# Autodesk Inventor assembly: Zlozenie
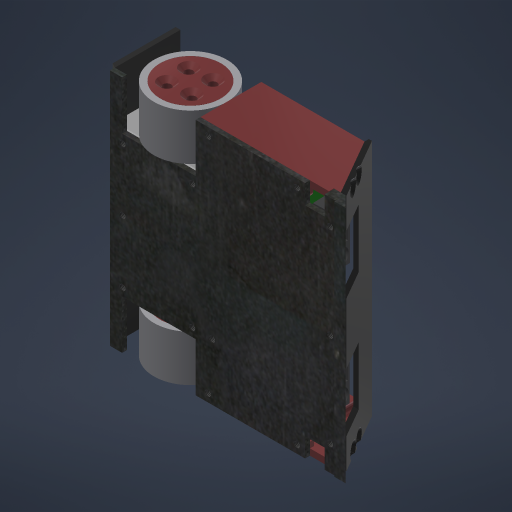
[picture p0: Inventor's stored thumbnail of the model, 512x512]
Saved by Autodesk Inventor 2023 (Build 270158000, 158)
## iProperties
Created: 2021-12-21
Part Number: Zlozenie
Material: Ogólny
Document SubType Name: Assembly
Designer: Michał
Mass: 427.985 g
Surface Area: 1162 cm^2
Volume: 132.956 cm^3
Density: 3.21899 g/cm^3
Author: Michał
## Documents named in this file (13)
- D:\Projekty\RoboIlo\Ser\3D\3D\Zlozenie.iam
- D:\Projekty\RoboIlo\Ser\3D\3D\Blacha.ipt
- D:\Projekty\RoboIlo\Ser\3D\3D\Plug2.ipt
- D:\Projekty\RoboIlo\Ser\3D\3D\Lewybok.ipt
- D:\Projekty\RoboIlo\Ser\3D\3D\Prawybok.ipt
- D:\Projekty\RoboIlo\Ser\3D\3D\Przod.ipt
- D:\Projekty\RoboIlo\Ser\3D\3D\Silnik.ipt
- D:\Projekty\RoboIlo\Ser\3D\3D\sds02a-with-sensor.ipt
- D:\Projekty\RoboIlo\Ser\3D\3D\Tyl.ipt
- D:\Projekty\RoboIlo\Ser\3D\3D\PrzekladniaLewa.iam
- D:\Projekty\RoboIlo\Ser\3D\3D\Kolo.iam
- D:\Projekty\RoboIlo\Ser\3D\3D\PrzekladniaPrawa.iam
- D:\Projekty\RoboIlo\Ser\3D\3D\Dach.ipt
## Components (15 placed, 12 different names)
1. Blacha:1 — Wstaw:1, Wstaw:2, Wstaw:19, Wstaw:20, Wstaw:21, Wstaw:22, Wstaw:36, Wstaw:37, Wstaw:43
2. Plug2:1 — Wstaw:1, Wstaw:2
3. Lewybok:1 — Wstaw:15, Zestawiający:9, Wstaw:19, Wstaw:20, Flush:1
4. Prawybok:1 — Wstaw:16, Zestawiający:10, Wstaw:17, Wstaw:18, Wstaw:21, Wstaw:22
5. Przod:1 — Wstaw:17, Wstaw:18
6. Silnik:1 — Wstaw:38, Wstaw:39
7. Silnik:2 — Wstaw:42
8. sds02a-with-sensor:1 — Wstaw:15, Zestawiający:9
9. sds02a-with-sensor:2 — Wstaw:16, Zestawiający:10
10. Tyl:1
11. PrzekladniaLewa:1 [sub-assembly] — Wstaw:36, Wstaw:37, Wstaw:38, Wstaw:39, Zestawiający:14, Zestawiający:15
12. Kolo:1 [sub-assembly] — Zestawiający:14, Zestawiający:15
13. PrzekladniaPrawa:1 [sub-assembly] — Wstaw:42, Wstaw:43, Zestawiający:16, Zestawiający:17
14. Kolo:2 [sub-assembly] — Zestawiający:16, Zestawiający:17
15. Dach:1 — Flush:1
## Relationships (23: Insert 16, Mate 6, Flush 1)
- Wstaw:1 [Insert]: Blacha:1 ↔ Plug2:1
- Wstaw:2 [Insert]: Blacha:1 ↔ Plug2:1
- Wstaw:15 [Insert]: Lewybok:1 ↔ sds02a-with-sensor:1
- Zestawiający:9 [Mate] (0.19 mm): Lewybok:1 ↔ sds02a-with-sensor:1
- Wstaw:16 [Insert]: Prawybok:1 ↔ sds02a-with-sensor:2
- Zestawiający:10 [Mate] (0.19 mm): Prawybok:1 ↔ sds02a-with-sensor:2
- Wstaw:17 [Insert]: Prawybok:1 ↔ Przod:1
- Wstaw:18 [Insert]: Prawybok:1 ↔ Przod:1
- Wstaw:19 [Insert]: Blacha:1 ↔ Lewybok:1
- Wstaw:20 [Insert]: Blacha:1 ↔ Lewybok:1
- Wstaw:21 [Insert]: Blacha:1 ↔ Prawybok:1
- Wstaw:22 [Insert]: Blacha:1 ↔ Prawybok:1
- Wstaw:36 [Insert]: Blacha:1 ↔ PrzekladniaLewa:1
- Wstaw:37 [Insert]: Blacha:1 ↔ PrzekladniaLewa:1
- Wstaw:38 [Insert]: Silnik:1 ↔ PrzekladniaLewa:1
- Wstaw:39 [Insert]: Silnik:1 ↔ PrzekladniaLewa:1
- Zestawiający:14 [Mate]: PrzekladniaLewa:1 ↔ Kolo:1
- Zestawiający:15 [Mate] (0.2 mm): PrzekladniaLewa:1 ↔ Kolo:1
- Wstaw:42 [Insert]: Silnik:2 ↔ PrzekladniaPrawa:1
- Wstaw:43 [Insert]: Blacha:1 ↔ PrzekladniaPrawa:1
- Zestawiający:16 [Mate] (0.2 mm): PrzekladniaPrawa:1 ↔ Kolo:2
- Zestawiający:17 [Mate]: PrzekladniaPrawa:1 ↔ Kolo:2
- Flush:1: Lewybok:1 ↔ Dach:1
